# Autodesk Inventor assembly: assembly_hoop
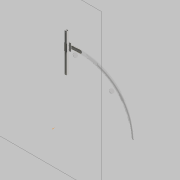
[picture p0: Inventor's stored thumbnail of the model, 180x180]
Saved by Autodesk Inventor 2021 (Build 250183000, 183)
## iProperties
Created: 2021-05-25
Part Number: assembly_hoop
Document SubType Name: Assembly
Designer: Watchdog
Author: Watchdog
## Documents named in this file (3)
- C:\Users\Watchdog\OneDrive - Flinders\Advn Mech Design Shared\6_Development\2_Design\inventor\assembly_hoop.iam
- C:\Users\Watchdog\OneDrive - Flinders\Advn Mech Design Shared\6_Development\2_Design\inventor\support\support_frameAssembly.iam
- C:\Users\Watchdog\OneDrive - Flinders\Advn Mech Design Shared\6_Development\2_Design\inventor\hoop_slider\hoops_sml_med_lrg.iam
## Components (2 placed, 2 different names)
1. support_frameAssembly:1 [sub-assembly] — Flush:1, Flush:2, Mate:1, Mate:4, Flush:3
2. hoops_sml_med_lrg:1 [sub-assembly] — Mate:4, Flush:3
## Relationships (5: Flush 3, Mate 2)
- Flush:1: support_frameAssembly:1
- Flush:2: support_frameAssembly:1
- Mate:1: support_frameAssembly:1
- Mate:4: support_frameAssembly:1 ↔ hoops_sml_med_lrg:1
- Flush:3: support_frameAssembly:1 ↔ hoops_sml_med_lrg:1
